# Autodesk Inventor assembly: Legassembly
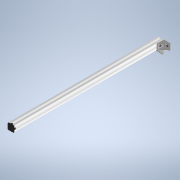
[picture p0: Inventor's stored thumbnail of the model, 180x180]
Saved by Autodesk Inventor 2020.2 (Build 242310000, 310)
## iProperties
Created: 2020-07-25
Part Number: Legassembly
Document SubType Name: Assembly
Designer: JK
Author: JK
## Documents named in this file (4)
- C:\Users\JK\Documents\Inventor\Mesa\Legassembly.iam
- C:\Users\JK\Documents\Inventor\Mesa\30x30x750.ipt
- C:\Users\JK\Documents\Inventor\Mesa\3030_endCap v4.ipt
- C:\Users\JK\Documents\Inventor\Mesa\Cornerassembly.iam
## Components (4 placed, 3 different names)
1. 30x30x750:1 — Mate:1, Flush:1, Flush:2, Mate:2, Flush:3, Mate:3, Flush:4, Flush:5
2. 3030_endCap v4:1 — Mate:1, Flush:1, Flush:2
3. Cornerassembly:1 [sub-assembly] — Mate:2, Flush:3
4. Cornerassembly:2 [sub-assembly] — Mate:3, Flush:4, Flush:5
## Relationships (8: Flush 5, Mate 3)
- Mate:1: 30x30x750:1 ↔ 3030_endCap v4:1
- Flush:1 (0.5 mm): 30x30x750:1 ↔ 3030_endCap v4:1
- Flush:2: 30x30x750:1 ↔ 3030_endCap v4:1
- Mate:2: 30x30x750:1 ↔ Cornerassembly:1
- Flush:3: 30x30x750:1 ↔ Cornerassembly:1
- Mate:3: 30x30x750:1 ↔ Cornerassembly:2
- Flush:4 (0.5 mm): 30x30x750:1 ↔ Cornerassembly:2
- Flush:5: 30x30x750:1 ↔ Cornerassembly:2
